# Autodesk Inventor assembly: PIP-Boy 6400 Mk_I Main Housing Back Subassembly
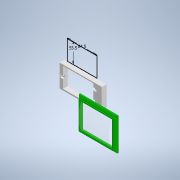
[picture p0: Inventor's stored thumbnail of the model, 180x180]
Saved by Autodesk Inventor 2021 (Build 250183000, 183)
## iProperties
Created: 2021-04-21
Part Number: PIP-Boy 6400 Mk_I Main Housing Back Subassembly
Document SubType Name: Assembly
Designer: trent
Author: trent
## Documents named in this file (5)
- C:\Users\trent\OneDrive - wmpenn.edu\Personal\PIP-Boy 6400 Mk.I\PIP-Boy 6400 Mk_I Main Housing Back Subassembly.iam
- C:\Users\trent\OneDrive - wmpenn.edu\Personal\PIP-Boy 6400 Mk.I\MainHousing_BackMainShell.ipt
- C:\Users\trent\OneDrive - wmpenn.edu\Personal\PIP-Boy 6400 Mk.I\MainHousing_FrontMainShell.ipt
- C:\Users\trent\OneDrive - wmpenn.edu\Personal\PIP-Boy 6400 Mk.I\MainHousing_Screen Acrylic.ipt
- C:\Users\trent\OneDrive - wmpenn.edu\Personal\PIP-Boy 6400 Mk.I\MainHousing_Screen Visor.ipt
## Components (4 placed, 4 different names)
1. MainHousing_BackMainShell:1
2. MainHousing_FrontMainShell:1
3. MainHousing_Screen Acrylic:1 — Mate:1, Mate:2, Mate:3
4. MainHousing_Screen Visor:1 — Mate:1, Mate:2, Mate:3
## Relationships (3: Mate 3)
- Mate:1: MainHousing_Screen Acrylic:1 ↔ MainHousing_Screen Visor:1
- Mate:2: MainHousing_Screen Acrylic:1 ↔ MainHousing_Screen Visor:1
- Mate:3: MainHousing_Screen Acrylic:1 ↔ MainHousing_Screen Visor:1
